# Autodesk Inventor assembly: CAD Model of Bridge Assembly
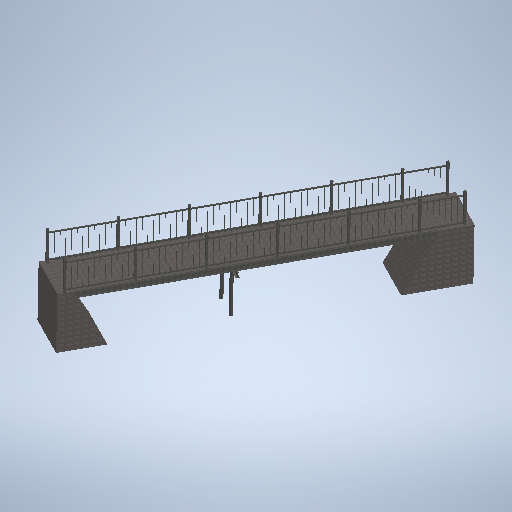
[picture p0: Inventor's stored thumbnail of the model, 512x512]
Saved by Autodesk Inventor 2025 (Build 290162000, 162)
## iProperties
Created: 2024-06-26
Part Number: CAD Model of Bridge Assembly
Document SubType Name: Assembly
Designer: track
Author: track
## Documents named in this file (10)
- C:\Users\track\OneDrive\Documents\USC-walking-bridges\Bridge_A\CAD_model\CAD Model of Bridge Assembly.iam
- C:\Users\track\OneDrive\Documents\USC-walking-bridges\Bridge_A\CAD_model\Concrete Walkway.ipt
- C:\Users\track\OneDrive\Documents\USC-walking-bridges\Bridge_A\CAD_model\Long I-Beam.ipt
- C:\Users\track\OneDrive\Documents\USC-walking-bridges\Bridge_A\CAD_model\Cylinder Supports.ipt
- C:\Users\track\OneDrive\Documents\USC-walking-bridges\Bridge_A\CAD_model\Short I-Beam.ipt
- C:\Users\track\OneDrive\Documents\USC-walking-bridges\Bridge_A\CAD_model\Cross Supports.ipt
- C:\Users\track\OneDrive\Documents\USC-walking-bridges\Bridge_A\CAD_model\Side near railing 1.ipt
- C:\Users\track\OneDrive\Documents\USC-walking-bridges\Bridge_A\CAD_model\Side near railing 7.ipt
- C:\Users\track\OneDrive\Documents\USC-walking-bridges\Bridge_A\CAD_model\Railing side A.ipt
- C:\Users\track\OneDrive\Documents\USC-walking-bridges\Bridge_A\CAD_model\Railing Side B.ipt
## Components (10 placed, 9 different names)
1. Concrete Walkway:1 — Mate:1, Mate:2, Flush:2, Flush:3, Flush:4, Flush:6, Mate:18, Flush:7, Flush:8, Mate:19, Flush:9, Flush:10, Mate:21, Mate:22, Mate:23, Mate:24, Mate:25, Mate:26, Mate:28, Mate:31
2. Long I-Beam:1 — Flush:1, Mate:4, Flush:3, Flush:6, Mate:18, Flush:7, Flush:8
3. Cylinder Supports:1 — Mate:5, Slider:1, Mate:17
4. Short I-Beam:1 — Flush:1, Mate:4, Flush:2, Mate:5, Slider:1, Mate:17
5. Cross Supports:1 — Mate:1, Mate:2, Mate:20
6. Long I-Beam:2 — Flush:4, Mate:19, Flush:9, Flush:10, Mate:20
7. Side near railing 1:1 — Mate:21, Mate:22, Mate:23, Mate:27, Mate:29, Mate:30, Mate:32
8. Side near railing 7:1 — Mate:24, Mate:25, Mate:26
9. Railing side A:1 — Mate:30, Mate:31, Mate:32
10. Railing Side B:1 — Mate:27, Mate:28, Mate:29
## Relationships (30: Mate 20, Flush 9, TranslationJoint 1)
- Mate:1 (381 mm): Concrete Walkway:1 ↔ Cross Supports:1
- Mate:2: Concrete Walkway:1 ↔ Cross Supports:1
- Flush:1 (-120.65 mm): Long I-Beam:1 ↔ Short I-Beam:1
- Mate:4: Long I-Beam:1 ↔ Short I-Beam:1
- Flush:2 (4724.4 mm): Concrete Walkway:1 ↔ Short I-Beam:1
- Mate:5: Cylinder Supports:1 ↔ Short I-Beam:1
- Flush:3: Concrete Walkway:1 ↔ Long I-Beam:1
- Flush:4: Concrete Walkway:1 ↔ Long I-Beam:2
- Flush:6: Concrete Walkway:1 ↔ Long I-Beam:1
- Slider:1 [TranslationJoint]: Cylinder Supports:1 ↔ Short I-Beam:1
- Mate:17 (-533.4 mm): Cylinder Supports:1 ↔ Short I-Beam:1
- Mate:18: Concrete Walkway:1 ↔ Long I-Beam:1
- Flush:7: Concrete Walkway:1 ↔ Long I-Beam:1
- Flush:8: Concrete Walkway:1 ↔ Long I-Beam:1
- Mate:19: Concrete Walkway:1 ↔ Long I-Beam:2
- Flush:9: Concrete Walkway:1 ↔ Long I-Beam:2
- Flush:10: Concrete Walkway:1 ↔ Long I-Beam:2
- Mate:20: Cross Supports:1 ↔ Long I-Beam:2
- Mate:21: Concrete Walkway:1 ↔ Side near railing 1:1
- Mate:22: Concrete Walkway:1 ↔ Side near railing 1:1
- Mate:23: Concrete Walkway:1 ↔ Side near railing 1:1
- Mate:24: Concrete Walkway:1 ↔ Side near railing 7:1
- Mate:25: Concrete Walkway:1 ↔ Side near railing 7:1
- Mate:26: Concrete Walkway:1 ↔ Side near railing 7:1
- Mate:27: Side near railing 1:1 ↔ Railing Side B:1
- Mate:28: Concrete Walkway:1 ↔ Railing Side B:1
- Mate:29 (203.2 mm): Side near railing 1:1 ↔ Railing Side B:1
- Mate:30: Side near railing 1:1 ↔ Railing side A:1
- Mate:31: Concrete Walkway:1 ↔ Railing side A:1
- Mate:32 (193.675 mm): Side near railing 1:1 ↔ Railing side A:1
